# Autodesk Inventor assembly: RT_FRM_V2_A_002_Dynamics
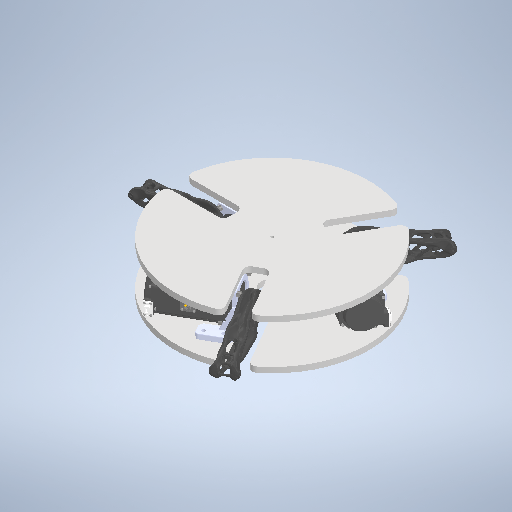
[picture p0: Inventor's stored thumbnail of the model, 512x512]
Saved by Autodesk Inventor 2025.3 (Build 293356000, 356)
## iProperties
Created: 2026-05-11
Part Number: RT_FRM_V2_A_002_Dynamics
Document SubType Name: Assembly
Designer: louis
Mass: 9176.21 g
Surface Area: 8073.41 cm^2
Volume: 2320.58 cm^3
Density: 3.95427 g/cm^3
Author: louis
## Documents named in this file (4)
- C:\Users\louis\OneDrive\Desktop\R_Trident\02_CAD\04_Subassemblies\RT_FRM_V2_A_002_Dynamics.iam
- C:\Users\louis\OneDrive\Desktop\R_Trident\02_CAD\03_Parts_Custom\RT_FRM_V2_MC_004_TopDynamicsPlate.ipt
- C:\Users\louis\OneDrive\Desktop\R_Trident\02_CAD\03_Parts_Custom\RT_FRM_V2_MC_004_BottomDynamicsPlate.ipt
- C:\Users\louis\OneDrive\Desktop\R_Trident\02_CAD\04_Subassemblies\RT_ARM_V2_A_001.iam
## Components (5 placed, 3 different names)
1. RT_FRM_V2_MC_004_TopDynamicsPlate:1 — Flush:1, Flush:2, Flush:3, Mate:1
2. RT_FRM_V2_MC_004_BottomDynamicsPlate:1 — Mate:1, Flush:4, Mate:2, Mate:3, Mate:4, Mate:5, Mate:6, Mate:7, Mate:8
3. RT_ARM_V2_A_001:1 [sub-assembly] — Mate:3, Mate:4
4. RT_ARM_V2_A_001:2 [sub-assembly] — Mate:5, Mate:6
5. RT_ARM_V2_A_001:3 [sub-assembly] — Mate:7, Mate:8
## Relationships (12: Mate 8, Flush 4)
- Flush:1: RT_FRM_V2_MC_004_TopDynamicsPlate:1
- Flush:2: RT_FRM_V2_MC_004_TopDynamicsPlate:1
- Flush:3: RT_FRM_V2_MC_004_TopDynamicsPlate:1
- Mate:1 (70 mm): RT_FRM_V2_MC_004_TopDynamicsPlate:1 ↔ RT_FRM_V2_MC_004_BottomDynamicsPlate:1
- Flush:4: RT_FRM_V2_MC_004_BottomDynamicsPlate:1
- Mate:2: RT_FRM_V2_MC_004_BottomDynamicsPlate:1
- Mate:3: RT_FRM_V2_MC_004_BottomDynamicsPlate:1 ↔ RT_ARM_V2_A_001:1
- Mate:4: RT_FRM_V2_MC_004_BottomDynamicsPlate:1 ↔ RT_ARM_V2_A_001:1
- Mate:5: RT_FRM_V2_MC_004_BottomDynamicsPlate:1 ↔ RT_ARM_V2_A_001:2
- Mate:6: RT_FRM_V2_MC_004_BottomDynamicsPlate:1 ↔ RT_ARM_V2_A_001:2
- Mate:7: RT_FRM_V2_MC_004_BottomDynamicsPlate:1 ↔ RT_ARM_V2_A_001:3
- Mate:8: RT_FRM_V2_MC_004_BottomDynamicsPlate:1 ↔ RT_ARM_V2_A_001:3
